# Autodesk Inventor assembly: Assembly ebeam heater IS v0
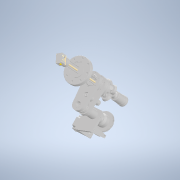
[picture p0: Inventor's stored thumbnail of the model, 180x180]
Saved by Autodesk Inventor 2020 (Build 240168000, 168)
## iProperties
Created: 2019-05-26
Part Number: Assembly ebeam heater IS v0
Document SubType Name: Assembly
Designer: isadmin
Author: isadmin
## Documents named in this file (16)
- C:\Users\ColinP\Documents\Inventor\INVENTOR IS_2019June01\Assembly ebeam heater IS v0.iam
- Assembly ebeam heater IS v0.iam
- C:\Users\ColinP\Documents\Inventor\INVENTOR IS_2019June01\block.ipt
- C:\Users\ColinP\Documents\Inventor\INVENTOR IS_2019June01\Shutter.ipt
- C:\Users\ColinP\Documents\Inventor\INVENTOR IS_2019June01\ceramic washer.ipt
- C:\Users\ColinP\Documents\Inventor\INVENTOR IS_2019June01\Shielding.ipt
- C:\Users\ColinP\Documents\Inventor\INVENTOR IS_2019June01\Bullet_v5_SiliconeSample.ipt
- C:\Users\ColinP\Documents\Inventor\INVENTOR IS_2019June01\Bullet_v5_SiliconeSample_TopPart.ipt
- C:\Users\ColinP\Documents\Inventor\INVENTOR IS_2019June01\670000.ipt
- C:\Users\ColinP\Documents\Inventor\INVENTOR IS_2019June01\MCF275-FlgMplxr-Cr1A5_(53-321020-A).ipt
- C:\Users\ColinP\Documents\Inventor\INVENTOR IS_2019June01\665501.ipt
- C:\Users\ColinP\Documents\Inventor\INVENTOR IS_2019June01\rotatable rod table.ipt
- C:\Users\ColinP\Documents\Inventor\igor\4.5 flange.ipt
- C:\Users\ColinP\Documents\Inventor\igor\square eyelet.ipt
- C:\Users\ColinP\Documents\Inventor\INVENTOR IS_2019June01\FlangeCF275 Bored_1112112 REV 1 .ipt
- C:\Users\ColinP\Documents\Inventor\igor\updated table+legs.iam
## Components (32 placed, 14 different names)
1. rotatable rod table:1 — Insert:6, Insert:9, Insert:22, Insert:23, Rotational:1, Insert:31, Insert:38, Rigid:1
2. block for bullet:1
3. Shutter:1
4. ceramic washer:1
5. ceramic washer:2
6. ceramic washer:3
7. ceramic washer:4
8. Shielding:1
9. ceramic washer:5
10. ceramic washer:6
11. ceramic washer:7
12. ceramic washer:8
13. Bullet_v5_SiliconeSample:1
14. Bullet_v5_SiliconeSample_TopPart:1
15. rotation_670000:1 — Insert:6, Rotational:1, Rigid:1
16. MCF275-FlgMplxr-Cr1A5_(53-321020-A):1
17. zstage_665501:1 — Insert:39
18. 4.5 flange:1 — Insert:9, Insert:23, Insert:24, Insert:25, Insert:26, Insert:27, Insert:28, Insert:29, Insert:30
19. updated table+legs:1 [sub-assembly] — Insert:22, Mate:23, Mate:24, Mate:25, Insert:38
20. square eyelet:1 — Insert:26, Mate:23
21. square eyelet:6 — Insert:29, Insert:30
22. square eyelet:7 — Insert:28
23. square eyelet:8 — Insert:27
24. square eyelet:9 — Insert:24
25. square eyelet:10 — Insert:25
26. FlangeCF275 Bored_1112112 REV 1 :1 — Insert:31, Insert:32, Insert:33, Insert:34, Insert:35, Insert:36, Insert:37, Insert:39
27. square eyelet:11 — Insert:36
28. square eyelet:12 — Insert:35
29. square eyelet:13 — Insert:37, Mate:24, Mate:25
30. square eyelet:14 — Insert:32
31. square eyelet:15 — Insert:34
32. square eyelet:16 — Insert:33
## Relationships (53: Mate 25, Insert 24, Flush 2, RevoluteJoint 1, WeldJoint 1)
- [Mate]: block for bullet:1 ↔ Shutter:1
- [Mate]: block for bullet:1 ↔ Shutter:1
- [Mate]: block for bullet:1 ↔ Shutter:1
- [Mate]: block for bullet:1 ↔ ceramic washer:2
- [Mate]: block for bullet:1 ↔ ceramic washer:2
- [Mate]: block for bullet:1 ↔ ceramic washer:1
- [Mate]: block for bullet:1 ↔ ceramic washer:1
- [Mate]: block for bullet:1 ↔ ceramic washer:4
- [Mate]: block for bullet:1 ↔ ceramic washer:4
- [Mate]: block for bullet:1 ↔ ceramic washer:3
- [Mate]: block for bullet:1 ↔ ceramic washer:3
- [Mate]: ceramic washer:1 ↔ Shielding:1
- [Flush]: block for bullet:1 ↔ Shielding:1
- [Flush]: block for bullet:1 ↔ Shielding:1
- [Mate]: block for bullet:1 ↔ ceramic washer:5
- [Mate]: block for bullet:1 ↔ ceramic washer:5
- [Mate]: block for bullet:1 ↔ ceramic washer:6
- [Mate]: block for bullet:1 ↔ ceramic washer:6
- [Mate]: block for bullet:1 ↔ ceramic washer:7
- [Mate]: block for bullet:1 ↔ ceramic washer:7
- [Mate]: block for bullet:1 ↔ ceramic washer:8
- [Mate]: block for bullet:1 ↔ ceramic washer:8
- [Mate] (0.0254 mm): Bullet_v5_SiliconeSample:1 ↔ Bullet_v5_SiliconeSample_TopPart:1
- [Mate]: Bullet_v5_SiliconeSample:1 ↔ Bullet_v5_SiliconeSample_TopPart:1
- [Insert]: block for bullet:1 ↔ Bullet_v5_SiliconeSample:1
- [Insert]: rotatable rod table:1 ↔ block for bullet:1
- [Insert]: rotatable rod table:1 ↔ block for bullet:1
- [Insert] (-0.254 mm): rotation_670000:1 ↔ MCF275-FlgMplxr-Cr1A5_(53-321020-A):1
- Insert:6: rotatable rod table:1 ↔ rotation_670000:1
- Insert:9 (101.6 mm): rotatable rod table:1 ↔ 4.5 flange:1
- Insert:22: rotatable rod table:1 ↔ updated table+legs:1
- Insert:23 (101.6 mm): rotatable rod table:1 ↔ 4.5 flange:1
- Insert:24: 4.5 flange:1 ↔ square eyelet:9
- Insert:25: 4.5 flange:1 ↔ square eyelet:10
- Insert:26: 4.5 flange:1 ↔ square eyelet:1
- Insert:27: 4.5 flange:1 ↔ square eyelet:8
- Insert:28: 4.5 flange:1 ↔ square eyelet:7
- Insert:29: 4.5 flange:1 ↔ square eyelet:6
- Insert:30: 4.5 flange:1 ↔ square eyelet:6
- Mate:23: updated table+legs:1 ↔ square eyelet:1
- Rotational:1 [RevoluteJoint]: rotatable rod table:1 ↔ rotation_670000:1
- Insert:31 (-43.18 mm): rotatable rod table:1 ↔ FlangeCF275 Bored_1112112 REV 1 :1
- Insert:32: FlangeCF275 Bored_1112112 REV 1 :1 ↔ square eyelet:14
- Insert:33: FlangeCF275 Bored_1112112 REV 1 :1 ↔ square eyelet:16
- Insert:34: FlangeCF275 Bored_1112112 REV 1 :1 ↔ square eyelet:15
- Insert:35: FlangeCF275 Bored_1112112 REV 1 :1 ↔ square eyelet:12
- Insert:36: FlangeCF275 Bored_1112112 REV 1 :1 ↔ square eyelet:11
- Insert:37: FlangeCF275 Bored_1112112 REV 1 :1 ↔ square eyelet:13
- Mate:24: updated table+legs:1 ↔ square eyelet:13
- Mate:25: updated table+legs:1 ↔ square eyelet:13
- Insert:38: rotatable rod table:1 ↔ updated table+legs:1
- Rigid:1 [WeldJoint]: rotatable rod table:1 ↔ rotation_670000:1
- Insert:39: zstage_665501:1 ↔ FlangeCF275 Bored_1112112 REV 1 :1
## Named parameters: d75_d58 = 0 mm, d76_d19 = 0 mm, d77_d22_d25 = 0 mm, d78_d23_d26 = 0 mm, d79_d24_d35 = 0 mm, d80_d25_d36 = 0 mm, d81_d26_d37 = 0 mm, d82_d27_d38 = 0 mm, d83_d28_d39 = 0 mm, d84_d29_d40 = 0 mm, d85_d30_d41 = 0 mm, d86_d31_d42 = 0 mm, d87_d43 = 0 mm, d88_d44 = 0 mm, d89_d45 = 0 mm, d90_d46 = 0 mm, d91_d47 = 0 mm, d92_d48 = 0 mm, d93_d49 = 0 mm, d94_d50 = 0 mm, d95_d51 = 0 mm, d96_d52 = 0 mm, d97_d53 = 0 mm, d98_d56_d0 = 0.0254 mm, d99_d57_d1 = 0 mm
